# Autodesk Inventor assembly: nerfbottomstack
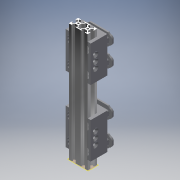
[picture p0: Inventor's stored thumbnail of the model, 180x180]
Saved by Autodesk Inventor 2018.3 (Build 223284000, 284)
## iProperties
Created: 2019-08-17
Part Number: nerfbottomstack
Document SubType Name: Assembly
Designer: Srinity
Author: Srinity
## Documents named in this file (5)
- C:\Users\Srinity\Documents\DIY Projects\NerfGun\nerfbottomstack.iam
- C:\Users\Srinity\Documents\DIY Projects\NerfGun\NerfBottomInsert.ipt
- C:\Users\Srinity\Documents\DIY Projects\NerfGun\NerfBottomStandoff.ipt
- C:\Users\Srinity\Documents\DIY Projects\NerfGun\V-Slot 20x40x1250 Linear Rail.ipt
- C:\Users\Srinity\Documents\DIY Projects\NerfGun\NerfRailMount.ipt
## Components (11 placed, 4 different names)
1. NerfBottomInsert:1 — Flush:1, Flush:2, Flush:3, Flush:4, Flush:6
2. NerfBottomStandoff:1 — Flush:1, Flush:7, Insert:8
3. V-Slot 20x40x1250 Linear Rail:1 — Flush:11, Mate:2, Mate:3, Mate:4, Mate:5
4. NerfBottomInsert:2 — Insert:5, Insert:6, Flush:3, Flush:5
5. NerfBottomStandoff:2 — Insert:5, Insert:6, Flush:9
6. NerfBottomInsert:3 — Insert:3, Insert:4, Flush:4, Flush:5, Flush:10
7. NerfBottomStandoff:3 — Insert:3, Insert:4, Flush:8, Flush:9, Flush:11, Insert:9
8. NerfBottomInsert:4 — Insert:1, Insert:2, Flush:2, Flush:6, Flush:10
9. NerfBottomStandoff:4 — Insert:1, Insert:2, Flush:7, Flush:8
10. NerfRailMount:1 — Mate:2, Mate:3, Insert:9
11. NerfRailMount:2 — Mate:4, Mate:5, Insert:8
## Relationships (23: Flush 11, Insert 8, Mate 4)
- Flush:1: NerfBottomInsert:1 ↔ NerfBottomStandoff:1
- Insert:1: NerfBottomInsert:4 ↔ NerfBottomStandoff:4
- Insert:2: NerfBottomInsert:4 ↔ NerfBottomStandoff:4
- Insert:3: NerfBottomInsert:3 ↔ NerfBottomStandoff:3
- Insert:4: NerfBottomInsert:3 ↔ NerfBottomStandoff:3
- Insert:5: NerfBottomInsert:2 ↔ NerfBottomStandoff:2
- Insert:6: NerfBottomInsert:2 ↔ NerfBottomStandoff:2
- Flush:2: NerfBottomInsert:1 ↔ NerfBottomInsert:4
- Flush:3: NerfBottomInsert:1 ↔ NerfBottomInsert:2
- Flush:4: NerfBottomInsert:1 ↔ NerfBottomInsert:3
- Flush:5 (40.5 mm): NerfBottomInsert:2 ↔ NerfBottomInsert:3
- Flush:6 (52.5 mm): NerfBottomInsert:1 ↔ NerfBottomInsert:4
- Flush:7: NerfBottomStandoff:1 ↔ NerfBottomStandoff:4
- Flush:8: NerfBottomStandoff:3 ↔ NerfBottomStandoff:4
- Flush:9: NerfBottomStandoff:2 ↔ NerfBottomStandoff:3
- Flush:10 (187 mm): NerfBottomInsert:3 ↔ NerfBottomInsert:4
- Flush:11 (-25.4 mm): V-Slot 20x40x1250 Linear Rail:1 ↔ NerfBottomStandoff:3
- Mate:2 (0.25 mm): V-Slot 20x40x1250 Linear Rail:1 ↔ NerfRailMount:1
- Mate:3 (0.25 mm): V-Slot 20x40x1250 Linear Rail:1 ↔ NerfRailMount:1
- Mate:4 (0.25 mm): V-Slot 20x40x1250 Linear Rail:1 ↔ NerfRailMount:2
- Mate:5 (0.25 mm): V-Slot 20x40x1250 Linear Rail:1 ↔ NerfRailMount:2
- Insert:8: NerfBottomStandoff:1 ↔ NerfRailMount:2
- Insert:9: NerfBottomStandoff:3 ↔ NerfRailMount:1
